# Autodesk Inventor assembly: CARCASA_ESTRUCTURA_Y_CHAPAS
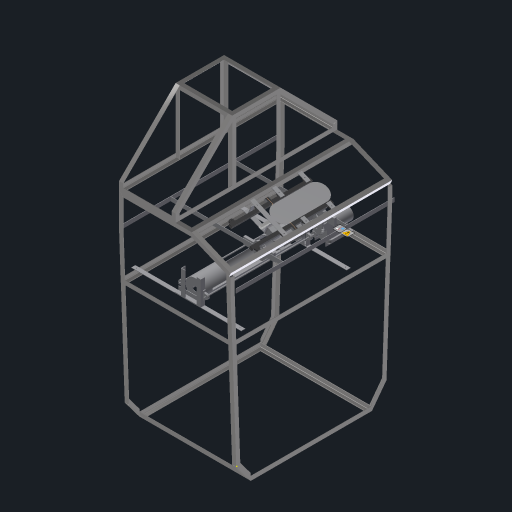
[picture p0: Inventor's stored thumbnail of the model, 512x512]
Saved by Autodesk Inventor 2024.3 (Build 283343000, 343)
## iProperties
Created: 2024-05-18
Part Number: CARCASA_ESTRUCTURA_Y_CHAPAS
Material: Generic
Document SubType Name: Assembly
Designer: Niler
Author: Niler
## Documents named in this file (6)
- C:\Users\Niler\OneDrive\Escritorio\RECICLADOR\RECICLADOR_MODELO_3D\VERSION_3_COMPLETA\CARCASA_ESTRUCTURA_Y_CHAPAS_1.iam
- C:\Users\Niler\OneDrive\Escritorio\RECICLADOR\RECICLADOR_MODELO_3D\VERSION_3_COMPLETA\ESTRUCTURA\ESTRUCTURA_COMPLETA.iam
- C:\Users\Niler\OneDrive\Escritorio\RECICLADOR\RECICLADOR_MODELO_3D\MECANISMO DE COMPACTADO\ENSAMBLE MECANISMO DE INGRESO.iam
- C:\Users\Niler\OneDrive\Escritorio\RECICLADOR\RECICLADOR_MODELO_3D\MECANISMO DE COMPACTADO\MECANISMO DE COMPACTADO.iam
- C:\Users\Niler\OneDrive\Escritorio\RECICLADOR\RECICLADOR_MODELO_3D\MECANISMO DE COMPACTADO\SEPARACION LATA-BOTELLA Y PAPEL.iam
- C:\Users\Niler\OneDrive\Escritorio\RECICLADOR\RECICLADOR_MODELO_3D\MECANISMO DE COMPACTADO\SOPORTE INERCIAL DE LA CAJA SEPARADORA.ipt
## Components (5 placed, 5 different names)
1. ESTRUCTURA_COMPLETA:1 [sub-assembly] — Mate:4, Mate:8, Mate:9, Mate:13, Mate:14, Mate:15
2. ENSAMBLE MECANISMO DE INGRESO:1 [sub-assembly] — Mate:14, Mate:15
3. MECANISMO DE COMPACTADO:1 [sub-assembly] — Mate:4, Mate:8
4. SEPARACION LATA-BOTELLA Y PAPEL:1 [sub-assembly] — Mate:9, Mate:12, Flush:1
5. SOPORTE INERCIAL DE LA CAJA SEPARADORA:1 — Mate:12, Mate:13, Flush:1
## Relationships (8: Mate 7, Flush 1)
- Mate:4: ESTRUCTURA_COMPLETA:1 ↔ MECANISMO DE COMPACTADO:1
- Mate:8 (50 mm): ESTRUCTURA_COMPLETA:1 ↔ MECANISMO DE COMPACTADO:1
- Mate:9 (220 mm): ESTRUCTURA_COMPLETA:1 ↔ SEPARACION LATA-BOTELLA Y PAPEL:1
- Mate:12: SEPARACION LATA-BOTELLA Y PAPEL:1 ↔ SOPORTE INERCIAL DE LA CAJA SEPARADORA:1
- Mate:13: ESTRUCTURA_COMPLETA:1 ↔ SOPORTE INERCIAL DE LA CAJA SEPARADORA:1
- Flush:1 (9.25 mm): SEPARACION LATA-BOTELLA Y PAPEL:1 ↔ SOPORTE INERCIAL DE LA CAJA SEPARADORA:1
- Mate:14: ESTRUCTURA_COMPLETA:1 ↔ ENSAMBLE MECANISMO DE INGRESO:1
- Mate:15: ESTRUCTURA_COMPLETA:1 ↔ ENSAMBLE MECANISMO DE INGRESO:1
